# Autodesk Inventor assembly: Rr.wing_assy
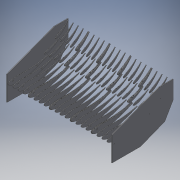
[picture p0: Inventor's stored thumbnail of the model, 180x180]
Saved by Autodesk Inventor 2018.2 (Build 222227000, 227)
## iProperties
Created: 2018-03-14
Part Number: Rr.wing_assy
Material: 一般
Document SubType Name: Assembly
Designer: ku_sk
Author: ku_sk
## Documents named in this file (5)
- C:\Users\ku_sk\Documents\Inventor\Aero\KS-15\Rr.wing\Rr.wing_assy.iam
- C:\Users\ku_sk\Documents\Inventor\Aero\KS-15\Rr.wing\parts\mainflap\mainflap.iam
- C:\Users\ku_sk\Documents\Inventor\Aero\KS-15\Rr.wing\parts\bracket1.ipt
- C:\Users\ku_sk\Documents\Inventor\Aero\KS-15\Rr.wing\parts\subflap\subflap.iam
- C:\Users\ku_sk\Documents\Inventor\Aero\KS-15\Rr.wing\parts\endplate.ipt
## Components (21 placed, 4 different names)
1. mainflap:1 [sub-assembly] — フラッシュ:1, メイト:1, 角度:1, メイト:2, メイト:3, メイト:4, メイト:5, メイト:6, メイト:7, メイト:9, メイト:10, メイト:12, メイト:13, メイト:18, メイト:19, メイト:24, メイト:25, メイト:57, メイト:61
2. mainflap:2 [sub-assembly] — メイト:8, メイト:9, メイト:10, メイト:20, メイト:21, メイト:22
3. mainflap:3 [sub-assembly] — メイト:11, メイト:12, メイト:13, メイト:14, メイト:16, メイト:17
4. mainflap:4 [sub-assembly] — メイト:23, メイト:24, メイト:25, メイト:56
5. mainflap:5 [sub-assembly] — メイト:15, メイト:18, メイト:19, メイト:60
6. subflap:1 [sub-assembly] — メイト:26, メイト:27, メイト:28
7. subflap:2 [sub-assembly] — メイト:29, メイト:30, メイト:31
8. subflap:3 [sub-assembly] — メイト:32, メイト:33, メイト:34, メイト:58, メイト:62
9. subflap:4 [sub-assembly] — メイト:35, メイト:36, メイト:37, メイト:39
10. subflap:5 [sub-assembly] — メイト:38, メイト:39, メイト:40
11. subflap:6 [sub-assembly] — メイト:41, メイト:42, メイト:43
12. subflap:7 [sub-assembly] — メイト:44, メイト:45, メイト:46
13. subflap:8 [sub-assembly] — メイト:47, メイト:48, メイト:49, メイト:59, メイト:63
14. subflap:9 [sub-assembly] — メイト:50, メイト:51, メイト:52
15. subflap:10 [sub-assembly] — メイト:53, メイト:54, メイト:55
16. bracket1:1 — メイト:20, メイト:21, メイト:22, メイト:23, メイト:26, メイト:27, メイト:28, メイト:29, メイト:30, メイト:31, メイト:41, メイト:42, メイト:43, メイト:44, メイト:45, メイト:46
17. bracket1:2 — メイト:5, メイト:6, メイト:7, メイト:8, メイト:32, メイト:33, メイト:34, メイト:47, メイト:48, メイト:49
18. bracket1:3 — メイト:2, メイト:3, メイト:4, メイト:11, メイト:35, メイト:36, メイト:37, メイト:50, メイト:51, メイト:52
19. bracket1:4 — メイト:14, メイト:15, メイト:16, メイト:17, メイト:38, メイト:40, メイト:53, メイト:54, メイト:55
20. endplate:1 — メイト:56, メイト:57, メイト:58, メイト:59
21. endplate:2 — メイト:60, メイト:61, メイト:62, メイト:63
## Relationships (65: Mate 63, Flush 1, Angle 1)
- フラッシュ:1 [Flush]: mainflap:1
- メイト:1 [Mate]: mainflap:1
- 角度:1 [Angle] (15 deg): mainflap:1
- メイト:2 [Mate]: mainflap:1 ↔ bracket1:3
- メイト:3 [Mate]: mainflap:1 ↔ bracket1:3
- メイト:4 [Mate]: mainflap:1 ↔ bracket1:3
- メイト:5 [Mate]: mainflap:1 ↔ bracket1:2
- メイト:6 [Mate]: mainflap:1 ↔ bracket1:2
- メイト:7 [Mate]: mainflap:1 ↔ bracket1:2
- メイト:8 [Mate]: mainflap:2 ↔ bracket1:2
- メイト:9 [Mate]: mainflap:1 ↔ mainflap:2
- メイト:10 [Mate]: mainflap:1 ↔ mainflap:2
- メイト:11 [Mate]: mainflap:3 ↔ bracket1:3
- メイト:12 [Mate]: mainflap:1 ↔ mainflap:3
- メイト:13 [Mate]: mainflap:1 ↔ mainflap:3
- メイト:14 [Mate]: mainflap:3 ↔ bracket1:4
- メイト:15 [Mate]: mainflap:5 ↔ bracket1:4
- メイト:16 [Mate]: mainflap:3 ↔ bracket1:4
- メイト:17 [Mate]: mainflap:3 ↔ bracket1:4
- メイト:18 [Mate]: mainflap:1 ↔ mainflap:5
- メイト:19 [Mate]: mainflap:1 ↔ mainflap:5
- メイト:20 [Mate]: mainflap:2 ↔ bracket1:1
- メイト:21 [Mate]: mainflap:2 ↔ bracket1:1
- メイト:22 [Mate]: mainflap:2 ↔ bracket1:1
- メイト:23 [Mate]: mainflap:4 ↔ bracket1:1
- メイト:24 [Mate]: mainflap:1 ↔ mainflap:4
- メイト:25 [Mate]: mainflap:1 ↔ mainflap:4
- メイト:26 [Mate]: subflap:1 ↔ bracket1:1
- メイト:27 [Mate]: subflap:1 ↔ bracket1:1
- メイト:28 [Mate]: subflap:1 ↔ bracket1:1
- メイト:29 [Mate]: subflap:2 ↔ bracket1:1
- メイト:30 [Mate]: subflap:2 ↔ bracket1:1
- メイト:31 [Mate]: subflap:2 ↔ bracket1:1
- メイト:32 [Mate]: subflap:3 ↔ bracket1:2
- メイト:33 [Mate]: subflap:3 ↔ bracket1:2
- メイト:34 [Mate]: subflap:3 ↔ bracket1:2
- メイト:35 [Mate]: subflap:4 ↔ bracket1:3
- メイト:36 [Mate]: subflap:4 ↔ bracket1:3
- メイト:37 [Mate]: subflap:4 ↔ bracket1:3
- メイト:38 [Mate]: subflap:5 ↔ bracket1:4
- メイト:39 [Mate]: subflap:4 ↔ subflap:5
- メイト:40 [Mate]: subflap:5 ↔ bracket1:4
- メイト:41 [Mate]: subflap:6 ↔ bracket1:1
- メイト:42 [Mate]: subflap:6 ↔ bracket1:1
- メイト:43 [Mate]: subflap:6 ↔ bracket1:1
- メイト:44 [Mate]: subflap:7 ↔ bracket1:1
- メイト:45 [Mate]: subflap:7 ↔ bracket1:1
- メイト:46 [Mate]: subflap:7 ↔ bracket1:1
- メイト:47 [Mate]: subflap:8 ↔ bracket1:2
- メイト:48 [Mate]: subflap:8 ↔ bracket1:2
- メイト:49 [Mate]: subflap:8 ↔ bracket1:2
- メイト:50 [Mate]: subflap:9 ↔ bracket1:3
- メイト:51 [Mate]: subflap:9 ↔ bracket1:3
- メイト:52 [Mate]: subflap:9 ↔ bracket1:3
- メイト:53 [Mate]: subflap:10 ↔ bracket1:4
- メイト:54 [Mate]: subflap:10 ↔ bracket1:4
- メイト:55 [Mate]: subflap:10 ↔ bracket1:4
- メイト:56 [Mate]: mainflap:4 ↔ endplate:1
- メイト:57 [Mate]: mainflap:1 ↔ endplate:1
- メイト:58 [Mate]: subflap:3 ↔ endplate:1
- メイト:59 [Mate]: subflap:8 ↔ endplate:1
- メイト:60 [Mate]: mainflap:5 ↔ endplate:2
- メイト:61 [Mate]: mainflap:1 ↔ endplate:2
- メイト:62 [Mate]: subflap:3 ↔ endplate:2
- メイト:63 [Mate]: subflap:8 ↔ endplate:2
